# Autodesk Inventor assembly: aluminium engine
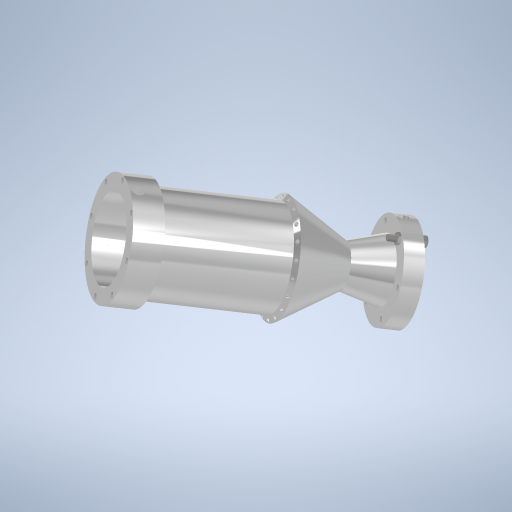
[picture p0: Inventor's stored thumbnail of the model, 512x512]
Saved by Autodesk Inventor 2023 (Build 270158000, 158)
## iProperties
Created: 2022-09-21
Part Number: aluminium engine
Document SubType Name: Assembly
Designer: station
Author: station
## Documents named in this file (6)
- C:\Users\station\Documents\Project\Liquid-engine-cooling-system\design files\ethanol engine 6\Aluminium engine\aluminium engine.iam
- C:\Users\station\Documents\Project\Liquid-engine-cooling-system\design files\ethanol engine 6\Aluminium engine\aluminium engine.ipt
- C:\Users\station\Documents\Project\Liquid-engine-cooling-system\design files\ethanol engine 6\Aluminium engine\back.ipt
- C:\Users\station\Documents\Inventor\Content Center Files\R2023\en-US\AS 1112 (4)\AS 1112 - M8(2).ipt
- C:\Users\station\Documents\Inventor\Content Center Files\R2023\en-US\AS 1427(02)\AS 1427 - M8 x 40(2).ipt
- C:\Users\station\Documents\Project\Liquid-engine-cooling-system\design files\ethanol engine 6\Aluminium engine\front.ipt
## Components (5 placed, 5 different names)
1. aluminium engine:1 — Mate:1, Mate:2, Mate:3, Mate:7, Mate:8, Mate:9, Mate:10
2. back:1 — Mate:1, Mate:2, Mate:3, Mate:4, Mate:5
3. AS 1427 - Metric M8 x 40:1 — Mate:4, Mate:5, Mate:6
4. AS 1112 (4) - Metric M8:1 — Mate:6, Mate:7
5. front:1 — Mate:8, Mate:9, Mate:10
## Relationships (10: Mate 10)
- Mate:1: aluminium engine:1 ↔ back:1
- Mate:2: aluminium engine:1 ↔ back:1
- Mate:3: aluminium engine:1 ↔ back:1
- Mate:4: back:1 ↔ AS 1427 - Metric M8 x 40:1
- Mate:5: back:1 ↔ AS 1427 - Metric M8 x 40:1
- Mate:6: AS 1427 - Metric M8 x 40:1 ↔ AS 1112 (4) - Metric M8:1
- Mate:7: aluminium engine:1 ↔ AS 1112 (4) - Metric M8:1
- Mate:8: aluminium engine:1 ↔ front:1
- Mate:9: aluminium engine:1 ↔ front:1
- Mate:10: aluminium engine:1 ↔ front:1
